# Autodesk Inventor assembly: B_shield_5
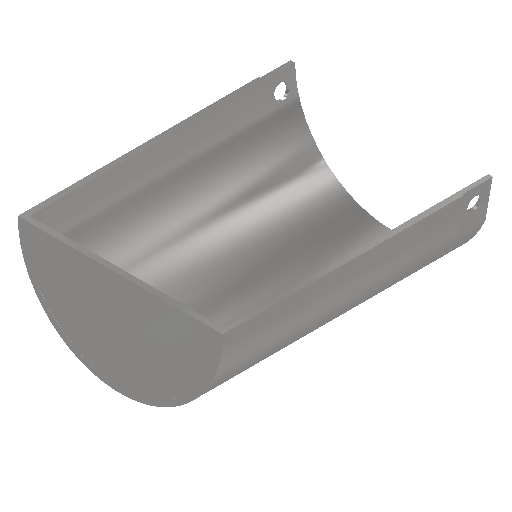
[picture p0: Inventor's stored thumbnail of the model, 512x512]
Saved by Autodesk Inventor 2026.2 (Build 302298000, 298)
## iProperties
Created: 2026-05-08
Part Number: B_shield_5
Document SubType Name: Assembly
Designer: zetsu
Author: zetsu
## Documents named in this file (3)
- C:\Users\mzts1\OneDrive - Kyoto University\ドキュメント\蓮尾研究室\3D_CAD\parts\BoronProbe\BoronProbe_5\parts\B_shield_5.iam
- C:\Users\mzts1\OneDrive - Kyoto University\ドキュメント\蓮尾研究室\3D_CAD\parts\BoronProbe\BoronProbe_5\parts\B_shield_5.ipt
- C:\Users\mzts1\OneDrive - Kyoto University\ドキュメント\蓮尾研究室\3D_CAD\parts\BoronProbe\BoronProbe_5\parts\B_shield_face_5.ipt
## Components (2 placed, 2 different names)
1. B_shield_5:1 — メイト:1, フラッシュ:1
2. B_shield_face_5:1 — メイト:1, フラッシュ:1
## Relationships (2: Mate 1, Flush 1)
- メイト:1 [Mate]: B_shield_5:1 ↔ B_shield_face_5:1
- フラッシュ:1 [Flush]: B_shield_5:1 ↔ B_shield_face_5:1
